# Autodesk Inventor assembly: ForeArmAssembly
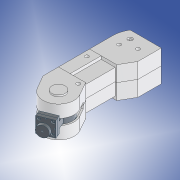
[picture p0: Inventor's stored thumbnail of the model, 180x180]
Saved by Autodesk Inventor 2017 (Build 210142000, 142)
## iProperties
Created: 2017-06-14
Part Number: ForeArmAssembly
Document SubType Name: Assembly
Designer: zallen
Author: zallen
## Documents named in this file (17)
- C:\Users\zallen\Documents\GitHub\cr-laundry-robot\src\Body\Arm Assembly\Bicep Assembly\BicepAssembly.iam
- C:\Users\zallen\Documents\GitHub\cr-laundry-robot\src\Body\Arm Assembly\Bicep Assembly\BA001.ipt
- C:\Users\zallen\Documents\GitHub\cr-laundry-robot\src\Body\Arm Assembly\Bicep Assembly\BA002.ipt
- C:\Users\zallen\Documents\GitHub\cr-laundry-robot\lib\Stepper Motor - NEMA 17\NEMA17.ipt
- C:\Users\zallen\Documents\GitHub\cr-laundry-robot\src\Body\Arm Assembly\Bicep Assembly\BA003.ipt
- C:\Users\zallen\Documents\GitHub\cr-laundry-robot\src\Body\Arm Assembly\Bicep Assembly\BA004.ipt
- C:\Users\zallen\Documents\GitHub\cr-laundry-robot\src\Body\Arm Assembly\Bicep Assembly\BA005.ipt
- C:\Users\zallen\Documents\GitHub\cr-laundry-robot\src\Body\Arm Assembly\Bicep Assembly\12 x 100mm Shaft.ipt
- C:\Users\zallen\Documents\GitHub\cr-laundry-robot\lib\6201RS\6201RS.ipt
- C:\Users\zallen\Documents\GitHub\cr-laundry-robot\src\Body\Arm Assembly\Bicep Assembly\BA007.ipt
- C:\Users\zallen\Documents\GitHub\cr-laundry-robot\src\Body\Arm Assembly\Bicep Assembly\BA008.ipt
- C:\Users\zallen\Documents\GitHub\cr-laundry-robot\src\Body\Arm Assembly\Bicep Assembly\BA011.ipt
- C:\Users\zallen\Documents\GitHub\cr-laundry-robot\src\Body\Arm Assembly\Bicep Assembly\BA010.ipt
- C:\Users\zallen\Documents\GitHub\cr-laundry-robot\src\Body\Arm Assembly\Bicep Assembly\10 x  80mm Shaft.ipt
- C:\Users\zallen\Documents\GitHub\cr-laundry-robot\src\Body\Arm Assembly\Bicep Assembly\BA012.ipt
- C:\Users\zallen\Documents\GitHub\cr-laundry-robot\src\Body\Arm Assembly\Bicep Assembly\BA013.ipt
- C:\Users\zallen\Documents\GitHub\cr-laundry-robot\src\Body\Arm Assembly\Bicep Assembly\BA014.ipt
## Components (19 placed, 16 different names)
1. BA001:1 — Mate:1, Mate:4, Mate:8, Mate:12, Mate:52, Mate:54, Mate:55, Mate:56, Mate:91, Mate:92, Mate:93, Mate:94, Mate:98, Mate:99
2. BA002:1 — Mate:1, Mate:4, Mate:53, Mate:57, Mate:98, Mate:99
3. BA003:1 — Mate:8, Mate:12, Mate:16, Mate:17, Mate:62, Mate:63, Mate:64, Mate:95, Mate:100, Mate:101
4. BA004:1 — Mate:44, Mate:72, Mate:83, Mate:104
5. BA005:1 — Mate:16, Mate:17, Mate:19, Mate:20, Mate:68, Mate:69
6. 12 x 100mm Shaft:1 — Mate:19, Mate:20, Mate:44, Mate:46, Mate:73, Mate:78
7. 6201RS:1 — Mate:78, Mate:82
8. 6201RS:2 — Mate:46, Mate:81
9. BA007:1 — Mate:84, Mate:85, Mate:86
10. BA008:1 — Mate:52, Mate:53, Mate:54
11. BA008:2 — Mate:55, Mate:56, Mate:57
12. BA011:1 — Rotation:4, Mate:95, Rotation:5, Mate:103
13. BA010:1 — Mate:62, Mate:63, Mate:64, Mate:72, Mate:102, Mate:103
14. 10 x  80mm Shaft:1 — Mate:68, Mate:69, Mate:70
15. BA012:1 — Mate:70, Rotation:3, Rotation:5, Mate:104
16. BA013:1 — Mate:73, Rotation:3, Mate:81, Mate:82, Mate:83, Mate:84, Mate:85, Mate:86
17. NEMA17:3 — Mate:89, Mate:91, Mate:92, Mate:93
18. BA014:1 — Mate:89, Rotation:4, Mate:94
19. 10 x  80mm Shaft:2 — Mate:100, Mate:101, Mate:102
## Relationships (47: Mate 44, RelateRotation 3)
- Mate:1: BA001:1 ↔ BA002:1
- Mate:4: BA001:1 ↔ BA002:1
- Mate:8: BA001:1 ↔ BA003:1
- Mate:12: BA001:1 ↔ BA003:1
- Mate:16: BA003:1 ↔ BA005:1
- Mate:17: BA003:1 ↔ BA005:1
- Mate:19: BA005:1 ↔ 12 x 100mm Shaft:1
- Mate:20: BA005:1 ↔ 12 x 100mm Shaft:1
- Mate:44: BA004:1 ↔ 12 x 100mm Shaft:1
- Mate:46: 12 x 100mm Shaft:1 ↔ 6201RS:2
- Mate:52: BA001:1 ↔ BA008:1
- Mate:53: BA002:1 ↔ BA008:1
- Mate:54: BA001:1 ↔ BA008:1
- Mate:55: BA001:1 ↔ BA008:2
- Mate:56: BA001:1 ↔ BA008:2
- Mate:57: BA002:1 ↔ BA008:2
- Mate:62: BA003:1 ↔ BA010:1
- Mate:63: BA003:1 ↔ BA010:1
- Mate:64: BA003:1 ↔ BA010:1
- Mate:68: BA005:1 ↔ 10 x  80mm Shaft:1
- Mate:69: BA005:1 ↔ 10 x  80mm Shaft:1
- Mate:70: 10 x  80mm Shaft:1 ↔ BA012:1
- Mate:72: BA004:1 ↔ BA010:1
- Mate:73: 12 x 100mm Shaft:1 ↔ BA013:1
- Rotation:3 [RelateRotation] (2 ul): BA012:1 ↔ BA013:1
- Mate:78: 12 x 100mm Shaft:1 ↔ 6201RS:1
- Mate:81: 6201RS:2 ↔ BA013:1
- Mate:82: 6201RS:1 ↔ BA013:1
- Mate:83: BA004:1 ↔ BA013:1
- Mate:84: BA007:1 ↔ BA013:1
- Mate:85: BA007:1 ↔ BA013:1
- Mate:86: BA007:1 ↔ BA013:1
- Mate:89: NEMA17:3 ↔ BA014:1
- Rotation:4 [RelateRotation] (25 ul): BA011:1 ↔ BA014:1
- Mate:91: BA001:1 ↔ NEMA17:3
- Mate:92: BA001:1 ↔ NEMA17:3
- Mate:93: BA001:1 ↔ NEMA17:3
- Mate:94: BA001:1 ↔ BA014:1
- Mate:95: BA003:1 ↔ BA011:1
- Rotation:5 [RelateRotation] (1 ul): BA011:1 ↔ BA012:1
- Mate:98: BA001:1 ↔ BA002:1
- Mate:99: BA001:1 ↔ BA002:1
- Mate:100: BA003:1 ↔ 10 x  80mm Shaft:2
- Mate:101: BA003:1 ↔ 10 x  80mm Shaft:2
- Mate:102: BA010:1 ↔ 10 x  80mm Shaft:2
- Mate:103: BA011:1 ↔ BA010:1
- Mate:104: BA004:1 ↔ BA012:1
